# Autodesk Inventor assembly: recovery_structure_asm
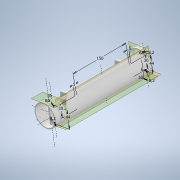
[picture p0: Inventor's stored thumbnail of the model, 180x180]
Saved by Autodesk Inventor 2020 (Build 240168000, 168)
## iProperties
Created: 2022-05-20
Part Number: recovery_structure_asm
Document SubType Name: Assembly
Designer: sp
Author: sp
## Documents named in this file (5)
- C:\Users\sp\Documents\Rocket\rocket\CAD\recovery_structure_asm.iam
- C:\Users\sp\Documents\Rocket\rocket\CAD\Verbindungsring_top.ipt
- C:\Users\sp\Documents\Rocket\rocket\CAD\Verbindungsring_bottom.ipt
- C:\Users\sp\Documents\Rocket\rocket\CAD\stange2.ipt
- C:\Users\sp\Documents\Rocket\rocket\CAD\Deckel_Parachute_4.ipt
## Components (5 placed, 4 different names)
1. Verbindungsring_top:1 — Einfügen:1, Einfügen:2, Einfügen:4
2. Verbindungsring_bottom:1 — Einfügen:3, Passend:1
3. stange2:1 — Einfügen:1, Passend:1
4. stange2:2 — Einfügen:2, Einfügen:3
5. Deckel_Parachute_4:1 — Einfügen:4
## Relationships (5: Insert 4, Mate 1)
- Einfügen:1 [Insert]: Verbindungsring_top:1 ↔ stange2:1
- Einfügen:2 [Insert]: Verbindungsring_top:1 ↔ stange2:2
- Einfügen:3 [Insert]: Verbindungsring_bottom:1 ↔ stange2:2
- Passend:1 [Mate]: Verbindungsring_bottom:1 ↔ stange2:1
- Einfügen:4 [Insert] (35 mm): Verbindungsring_top:1 ↔ Deckel_Parachute_4:1
